# Autodesk Inventor assembly: Test Fit Assembly
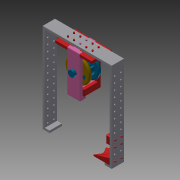
[picture p0: Inventor's stored thumbnail of the model, 180x180]
Saved by Autodesk Inventor 2015 (Build 190159000, 159)
## iProperties
Created: 2016-11-23
Part Number: Test Fit Assembly
Document SubType Name: Assembly
Designer: Markus
Author: Markus
## Documents named in this file (8)
- C:\Users\Markus\Documents\Inventor\Project IRIS\Test Fit Assembly.iam
- C:\Users\Markus\Documents\Inventor\Project IRIS\Bay Door Prototype Mk1.ipt
- C:\Users\Markus\Documents\Inventor\Project IRIS\Bottom Pivot Mk1.ipt
- C:\Users\Markus\Documents\Inventor\Project IRIS\Short Brace Prototype Mk1.ipt
- C:\Users\Markus\Documents\Inventor\Project IRIS\Spool Holder Main Section Mk1.ipt
- C:\Users\Markus\Documents\Inventor\Project IRIS\Spool Main Section Mk1.ipt
- C:\Users\Markus\Documents\Inventor\Project IRIS\Spool Cap Section Mk1.ipt
- C:\Users\Markus\Documents\Inventor\Project IRIS\Spool Holder Cap Section Mk1.ipt
## Components (7 placed, 7 different names)
1. Bay Door Prototype Mk1:1 — Mate:1, Flush:1, Mate:2, Mate:3, Insert:1, Mate:4, Mate:5, Insert:2, Insert:3, Insert:6
2. Bottom Pivot Mk1:1 — Mate:1, Flush:1, Mate:2
3. Short Brace Prototype Mk1:1 — Mate:3, Insert:1, Mate:4
4. Spool Holder Main Section Mk1:1 — Mate:5, Insert:2, Insert:3, Insert:4, Flush:2, Mate:7
5. Spool Main Section Mk1:1 — Insert:4, Mate:6, Insert:5, Angle:1
6. Spool Cap Section Mk1:1 — Mate:6, Insert:5, Angle:1
7. Spool Holder Cap Section Mk1:1 — Flush:2, Mate:7, Insert:6
## Relationships (16: Mate 7, Insert 6, Flush 2, Angle 1)
- Mate:1: Bay Door Prototype Mk1:1 ↔ Bottom Pivot Mk1:1
- Flush:1: Bay Door Prototype Mk1:1 ↔ Bottom Pivot Mk1:1
- Mate:2: Bay Door Prototype Mk1:1 ↔ Bottom Pivot Mk1:1
- Mate:3: Bay Door Prototype Mk1:1 ↔ Short Brace Prototype Mk1:1
- Insert:1: Bay Door Prototype Mk1:1 ↔ Short Brace Prototype Mk1:1
- Mate:4: Bay Door Prototype Mk1:1 ↔ Short Brace Prototype Mk1:1
- Mate:5: Bay Door Prototype Mk1:1 ↔ Spool Holder Main Section Mk1:1
- Insert:2: Bay Door Prototype Mk1:1 ↔ Spool Holder Main Section Mk1:1
- Insert:3: Bay Door Prototype Mk1:1 ↔ Spool Holder Main Section Mk1:1
- Insert:4 (1.27 mm): Spool Holder Main Section Mk1:1 ↔ Spool Main Section Mk1:1
- Mate:6: Spool Main Section Mk1:1 ↔ Spool Cap Section Mk1:1
- Insert:5: Spool Main Section Mk1:1 ↔ Spool Cap Section Mk1:1
- Angle:1 (0 deg): Spool Main Section Mk1:1 ↔ Spool Cap Section Mk1:1
- Flush:2: Spool Holder Main Section Mk1:1 ↔ Spool Holder Cap Section Mk1:1
- Mate:7: Spool Holder Main Section Mk1:1 ↔ Spool Holder Cap Section Mk1:1
- Insert:6: Bay Door Prototype Mk1:1 ↔ Spool Holder Cap Section Mk1:1
